# Autodesk Inventor assembly: WheelAssembly3.0
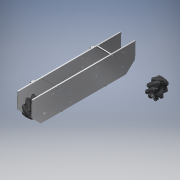
[picture p0: Inventor's stored thumbnail of the model, 180x180]
Saved by Autodesk Inventor 2019 (Build 230136000, 136)
## iProperties
Created: 2017-07-22
Part Number: WheelAssembly3.0
Document SubType Name: Assembly
Designer: User
Mass: 2301.48 g
Surface Area: 4071.67 cm^2
Volume: 902.346 cm^3
Density: 2.55055 g/cm^3
Author: User
## Documents named in this file (23)
- C:\Robotics\CAD\2020-21-CAD\Drivetrain\InvertedDriveTrain.iam
- C:\Robotics\CAD\COTSParts\Tetrix\tetrix-motor-mounts-1.snapshot.1\Tetrex 2pc motor mount.ipt
- C:\Robotics\CAD\COTSParts\Actobotics\615 parts\615398.25inBoreBeveledGears.ipt
- C:\Robotics\CAD\2016-17_CAD\Custom COTS\4inax.ipt
- C:\Robotics\CAD\COTSParts\Wheels\4in Wheel Intergreated Hub 8mm Rev2.ipt
- C:\Robotics\CAD\COTSParts\Actobotics\Thrust Bearings\6655K13.ipt
- C:\Robotics\CAD\2018-19_CAD\Offseason\InvertedDrivePlateOutside.ipt
- C:\Robotics\CAD\2018-19_CAD\Offseason\InvertedDrivePlateInside.ipt
- C:\Robotics\CAD\COTSParts\Actobotics\535 parts\535198Bearing.25ID.5OD.ipt
- C:\Robotics\CAD\2018-19_CAD\Offseason\MotorFixedPositionMountInvertedDrive.ipt
- C:\Robotics\CAD\COTSParts\Actobotics\Collar.ipt
- C:\Robotics\CAD\COTSParts\Fasteners\6-32 SHCS x500.ipt
- C:\Robotics\CAD\COTSParts\Fasteners\Hex Standoff 6-32 x2250.ipt
- C:\Robotics\CAD\COTSParts\Motors\am-3102NeveRest20 (1).ipt
- C:\Robotics\CAD\COTSParts\Tetrix\tetrix-motor-mounts-1.snapshot.1\Tetrex 2pc motor mount_MIR.ipt
- C:\Robotics\CAD\COTSParts\Actobotics\615 parts\615398.25inBoreBeveledGears_MIR.ipt
- C:\Robotics\CAD\COTSParts\Actobotics\Thrust Bearings\6655K13_MIR.ipt
- C:\Robotics\CAD\COTSParts\Actobotics\535 parts\535198Bearing.25ID.5OD_MIR.ipt
- C:\Robotics\CAD\2018-19_CAD\Offseason\MotorFixedPositionMountInvertedDrive_MIR.ipt
- C:\Robotics\CAD\COTSParts\Fasteners\6-32 SHCS x500_MIR.ipt
- C:\Robotics\CAD\COTSParts\Motors\am-3102NeveRest20 (1)_MIR.ipt
- C:\Robotics\CAD\COTSParts\Rev\REV-41-1656MecanumWheel.iam
- C:\Robotics\CAD\COTSParts\Rev\REV-41-1657MecanumWheelRight.iam
## Components (43 placed, 22 different names)
1. Tetrex 2pc motor mount:1 — Insert:84, Flush:5, Mate:42, Mate:43, Flush:6, Flush:8
2. 615398.25inBoreBeveledGears:2 — Insert:47, Mate:35, Mate:40, Rotation:6
3. 615398.25inBoreBeveledGears:3 — Insert:77, Mate:40, Mate:45, Rotation:6
4. 4inax:4 — Insert:147, Mate:45, Mate:63
5. 4in Wheel Intergreated Hub 8mm Rev2:1
6. 4in Wheel Intergreated Hub 8mm Rev2:2
7. 6655K13:2 — Insert:77, Mate:44
8. 6655K13:4 — Insert:47, Mate:36
9. InvertedDrivePlateOutside:1 — Insert:71, Insert:74, Insert:128, Insert:129, Insert:130, Insert:131, Insert:136, Insert:137, Insert:138, Insert:139, Symmetry:1
10. InvertedDrivePlateInside:1 — Insert:90, Insert:132, Insert:133, Insert:134, Insert:135, Insert:140, Insert:141, Insert:142, Insert:143, Mate:43, Flush:6, Mate:44, Symmetry:1, Mate:52, Mate:56, Mate:57, Mate:60, Mate:61
11. 535198Bearing.25ID.5OD:1 — Insert:71, Insert:86
12. 535198Bearing.25ID.5OD:2 — Insert:74, Mate:58, Flush:9
13. MotorFixedPositionMountInvertedDrive:1 — Insert:84, Insert:120, Insert:121, Mate:35, Mate:36, Mate:37
14. Collar:1 — Insert:86, Insert:147
15. 535198Bearing.25ID.5OD:5 — Insert:90
16. 6-32 SHCS x500:14 — Insert:120
17. 6-32 SHCS x500:15 — Insert:121
18. Hex Standoff 6-32 x2250:1 — Insert:129, Insert:134
19. Hex Standoff 6-32 x2250:2 — Insert:128, Insert:132
20. Hex Standoff 6-32 x2250:3 — Insert:131, Insert:135
21. Hex Standoff 6-32 x2250:4 — Insert:130, Insert:133
22. 6-32 SHCS x500:22 — Insert:136
23. 6-32 SHCS x500:23 — Insert:137
24. 6-32 SHCS x500:24 — Insert:138
25. 6-32 SHCS x500:25 — Insert:139
26. 6-32 SHCS x500:26 — Insert:140
27. 6-32 SHCS x500:27 — Insert:141
28. 6-32 SHCS x500:28 — Insert:142
29. 6-32 SHCS x500:29 — Insert:143
30. am-3102NeveRest20 (1):1 — Mate:37, Flush:5, Mate:42
31. Tetrex 2pc motor mount_MIR:1 — Insert:150, Mate:50, Flush:7, Flush:8, Mate:52, Mate:53
32. 615398.25inBoreBeveledGears_MIR:1 — Rotation:7, Mate:46, Insert:149, Mate:49
33. 615398.25inBoreBeveledGears_MIR:2 — Rotation:7, Mate:46, Insert:148, Mate:62
34. 6655K13_MIR:1 — Insert:148, Mate:59
35. 6655K13_MIR:2 — Insert:149, Mate:48
36. 535198Bearing.25ID.5OD_MIR:1 — Mate:56, Mate:59, Mate:60, Mate:61
37. MotorFixedPositionMountInvertedDrive_MIR:1 — Mate:48, Mate:49, Insert:150, Insert:153, Insert:154, Mate:51
38. 6-32 SHCS x500_MIR:1 — Insert:153
39. 6-32 SHCS x500_MIR:2 — Insert:154
40. am-3102NeveRest20 (1)_MIR:1 — Mate:50, Flush:7, Mate:51
41. 4inax:5 — Mate:57, Mate:58, Flush:9, Mate:62, Mate:64
42. REV-41-1656MecanumWheel:1 [sub-assembly] — Mate:64
43. REV-41-1657MecanumWheelRight:1 [sub-assembly] — Mate:63
## Relationships (63: Insert 31, Mate 24, Flush 5, RelateRotation 2, Symmetry 1)
- Insert:47: 615398.25inBoreBeveledGears:2 ↔ 6655K13:4
- Insert:71: InvertedDrivePlateOutside:1 ↔ 535198Bearing.25ID.5OD:1
- Insert:74: InvertedDrivePlateOutside:1 ↔ 535198Bearing.25ID.5OD:2
- Insert:77: 615398.25inBoreBeveledGears:3 ↔ 6655K13:2
- Insert:84: Tetrex 2pc motor mount:1 ↔ MotorFixedPositionMountInvertedDrive:1
- Insert:86: 535198Bearing.25ID.5OD:1 ↔ Collar:1
- Insert:90: InvertedDrivePlateInside:1 ↔ 535198Bearing.25ID.5OD:5
- Insert:120: MotorFixedPositionMountInvertedDrive:1 ↔ 6-32 SHCS x500:14
- Insert:121: MotorFixedPositionMountInvertedDrive:1 ↔ 6-32 SHCS x500:15
- Insert:128: InvertedDrivePlateOutside:1 ↔ Hex Standoff 6-32 x2250:2
- Insert:129: InvertedDrivePlateOutside:1 ↔ Hex Standoff 6-32 x2250:1
- Insert:130: InvertedDrivePlateOutside:1 ↔ Hex Standoff 6-32 x2250:4
- Insert:131: InvertedDrivePlateOutside:1 ↔ Hex Standoff 6-32 x2250:3
- Insert:132: InvertedDrivePlateInside:1 ↔ Hex Standoff 6-32 x2250:2
- Insert:133: InvertedDrivePlateInside:1 ↔ Hex Standoff 6-32 x2250:4
- Insert:134: InvertedDrivePlateInside:1 ↔ Hex Standoff 6-32 x2250:1
- Insert:135: InvertedDrivePlateInside:1 ↔ Hex Standoff 6-32 x2250:3
- Insert:136: InvertedDrivePlateOutside:1 ↔ 6-32 SHCS x500:22
- Insert:137: InvertedDrivePlateOutside:1 ↔ 6-32 SHCS x500:23
- Insert:138: InvertedDrivePlateOutside:1 ↔ 6-32 SHCS x500:24
- Insert:139: InvertedDrivePlateOutside:1 ↔ 6-32 SHCS x500:25
- Insert:140: InvertedDrivePlateInside:1 ↔ 6-32 SHCS x500:26
- Insert:141: InvertedDrivePlateInside:1 ↔ 6-32 SHCS x500:27
- Insert:142: InvertedDrivePlateInside:1 ↔ 6-32 SHCS x500:28
- Insert:143: InvertedDrivePlateInside:1 ↔ 6-32 SHCS x500:29
- Insert:147: 4inax:4 ↔ Collar:1
- Mate:35: 615398.25inBoreBeveledGears:2 ↔ MotorFixedPositionMountInvertedDrive:1
- Mate:36: 6655K13:4 ↔ MotorFixedPositionMountInvertedDrive:1
- Mate:37: MotorFixedPositionMountInvertedDrive:1 ↔ am-3102NeveRest20 (1):1
- Flush:5: Tetrex 2pc motor mount:1 ↔ am-3102NeveRest20 (1):1
- Mate:40 (-7.6197 mm): 615398.25inBoreBeveledGears:2 ↔ 615398.25inBoreBeveledGears:3
- Mate:42: Tetrex 2pc motor mount:1 ↔ am-3102NeveRest20 (1):1
- Mate:43: Tetrex 2pc motor mount:1 ↔ InvertedDrivePlateInside:1
- Flush:6 (25.4 mm): Tetrex 2pc motor mount:1 ↔ InvertedDrivePlateInside:1
- Mate:44: 6655K13:2 ↔ InvertedDrivePlateInside:1
- Mate:45: 615398.25inBoreBeveledGears:3 ↔ 4inax:4
- Rotation:6 [RelateRotation] (1 ul): 615398.25inBoreBeveledGears:2 ↔ 615398.25inBoreBeveledGears:3
- Symmetry:1: InvertedDrivePlateOutside:1 ↔ InvertedDrivePlateInside:1
- Rotation:7 [RelateRotation] (1 ul): 615398.25inBoreBeveledGears_MIR:1 ↔ 615398.25inBoreBeveledGears_MIR:2
- Mate:46 (-7.6197 mm): 615398.25inBoreBeveledGears_MIR:1 ↔ 615398.25inBoreBeveledGears_MIR:2
- Insert:148: 615398.25inBoreBeveledGears_MIR:2 ↔ 6655K13_MIR:1
- Insert:149: 615398.25inBoreBeveledGears_MIR:1 ↔ 6655K13_MIR:2
- Mate:48: 6655K13_MIR:2 ↔ MotorFixedPositionMountInvertedDrive_MIR:1
- Mate:49: 615398.25inBoreBeveledGears_MIR:1 ↔ MotorFixedPositionMountInvertedDrive_MIR:1
- Insert:150: Tetrex 2pc motor mount_MIR:1 ↔ MotorFixedPositionMountInvertedDrive_MIR:1
- Insert:153: MotorFixedPositionMountInvertedDrive_MIR:1 ↔ 6-32 SHCS x500_MIR:1
- Insert:154: MotorFixedPositionMountInvertedDrive_MIR:1 ↔ 6-32 SHCS x500_MIR:2
- Mate:50: Tetrex 2pc motor mount_MIR:1 ↔ am-3102NeveRest20 (1)_MIR:1
- Flush:7: Tetrex 2pc motor mount_MIR:1 ↔ am-3102NeveRest20 (1)_MIR:1
- Mate:51: MotorFixedPositionMountInvertedDrive_MIR:1 ↔ am-3102NeveRest20 (1)_MIR:1
- Flush:8: Tetrex 2pc motor mount:1 ↔ Tetrex 2pc motor mount_MIR:1
- Mate:52: InvertedDrivePlateInside:1 ↔ Tetrex 2pc motor mount_MIR:1
- Mate:53 (122.8344 mm): Tetrex 2pc motor mount_MIR:1
- Mate:56: InvertedDrivePlateInside:1 ↔ 535198Bearing.25ID.5OD_MIR:1
- Mate:57: InvertedDrivePlateInside:1 ↔ 4inax:5
- Mate:58: 535198Bearing.25ID.5OD:2 ↔ 4inax:5
- Flush:9: 535198Bearing.25ID.5OD:2 ↔ 4inax:5
- Mate:59: 6655K13_MIR:1 ↔ 535198Bearing.25ID.5OD_MIR:1
- Mate:60: InvertedDrivePlateInside:1 ↔ 535198Bearing.25ID.5OD_MIR:1
- Mate:61: InvertedDrivePlateInside:1 ↔ 535198Bearing.25ID.5OD_MIR:1
- Mate:62: 615398.25inBoreBeveledGears_MIR:2 ↔ 4inax:5
- Mate:63: 4inax:4 ↔ REV-41-1657MecanumWheelRight:1
- Mate:64: 4inax:5 ↔ REV-41-1656MecanumWheel:1
